# Autodesk Inventor assembly: 01 Gesamtsystem
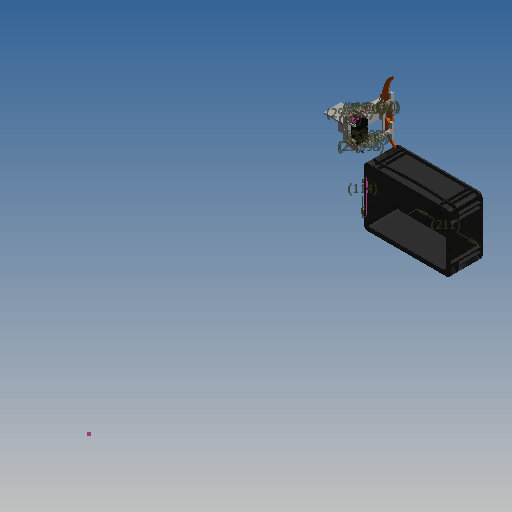
[picture p0: Inventor's stored thumbnail of the model, 512x512]
Saved by Autodesk Inventor 2026.2 (Build 302298000, 298)
## iProperties
Part Number: 01 Gesamtsystem
Document SubType Name: Baugruppe
Designer: Schally
Author: Schally
## Documents named in this file (11)
- E:\06 Carologistics\02 Zeichnungen Greifer System\01 Gesamtsystem.iam
- E:\06 Carologistics\02 Zeichnungen Greifer System\01-01 Gripper_Basis_2 Servo System.ipt
- E:\06 Carologistics\02 Zeichnungen Greifer System\01-02-01 Sandard-Servo.ipt
- E:\06 Carologistics\02 Zeichnungen Greifer System\01-02-03 Gripper neu rechts.ipt
- E:\06 Carologistics\02 Zeichnungen Greifer System\01-03-01 Zange Links.iam
- E:\06 Carologistics\02 Zeichnungen Greifer System\01-03-02 Zange rechts.iam
- E:\06 Carologistics\02 Zeichnungen Greifer System\01-03-05 Muttern.ipt
- E:\06 Carologistics\02 Zeichnungen Greifer System\01-03-06 Schraube unten.ipt
- E:\06 Carologistics\02 Zeichnungen Greifer System\01-05 Absicherung Richtung Kugellager.ipt
- E:\06 Carologistics\02 Zeichnungen Greifer System\00 Zeichnung Box.ipt
- E:\06 Carologistics\02 Zeichnungen Greifer System\01-02-02 Gripper neu links.ipt
## Components (14 placed, 10 different names)
1. 01-01 Gripper_Basis_2 Servo System:1 — Einfügen:1, Passend:1, Passend:20, Passend:21, Passend:22, Passend:23, Passend:24, Passend:25, Passend:28
2. 01-02-01 Sandard-Servo:1 — Passend:20, Passend:21, Passend:22, Passend:26
3. 01-02-03 Gripper neu rechts:1 — Passend:26
4. 01-03-01 Zange Links:1 [sub-assembly] — Passend:3, Passend:5, Passend:9
5. 01-03-02 Zange rechts:1 [sub-assembly] — Passend:2, Passend:10, Passend:11
6. 01-03-05 Muttern:1 — Passend:4, Passend:5
7. 01-03-06 Schraube unten:1 — Einfügen:2, Passend:2, Passend:3, Passend:4, Passend:6, Passend:7, Passend:8, Passend:12
8. 01-05 Absicherung Richtung Kugellager:1 — Einfügen:1, Passend:1, Einfügen:2
9. 01-03-05 Muttern:2 — Passend:8, Passend:11, Passend:12
10. 01-03-05 Muttern:3 — Passend:6, Passend:10, Passend:13
11. 01-03-05 Muttern:4 — Passend:7, Passend:9, Passend:13
12. 00 Zeichnung Box:1 — Passend:28
13. 01-02-01 Sandard-Servo:2 — Passend:23, Passend:24, Passend:25, Passend:27
14. 01-02-02 Gripper neu links:1 — Passend:27
## Relationships (24: Mate 22, Insert 2)
- Einfügen:1 [Insert]: 01-01 Gripper_Basis_2 Servo System:1 ↔ 01-05 Absicherung Richtung Kugellager:1
- Passend:1 [Mate]: 01-01 Gripper_Basis_2 Servo System:1 ↔ 01-05 Absicherung Richtung Kugellager:1
- Einfügen:2 [Insert]: 01-03-06 Schraube unten:1 ↔ 01-05 Absicherung Richtung Kugellager:1
- Passend:2 [Mate]: 01-03-02 Zange rechts:1 ↔ 01-03-06 Schraube unten:1
- Passend:3 [Mate]: 01-03-01 Zange Links:1 ↔ 01-03-06 Schraube unten:1
- Passend:4 [Mate]: 01-03-05 Muttern:1 ↔ 01-03-06 Schraube unten:1
- Passend:5 [Mate]: 01-03-01 Zange Links:1 ↔ 01-03-05 Muttern:1
- Passend:6 [Mate]: 01-03-06 Schraube unten:1 ↔ 01-03-05 Muttern:3
- Passend:7 [Mate]: 01-03-06 Schraube unten:1 ↔ 01-03-05 Muttern:4
- Passend:8 [Mate]: 01-03-06 Schraube unten:1 ↔ 01-03-05 Muttern:2
- Passend:9 [Mate]: 01-03-01 Zange Links:1 ↔ 01-03-05 Muttern:4
- Passend:10 [Mate]: 01-03-02 Zange rechts:1 ↔ 01-03-05 Muttern:3
- Passend:11 [Mate]: 01-03-02 Zange rechts:1 ↔ 01-03-05 Muttern:2
- Passend:12 [Mate]: 01-03-06 Schraube unten:1 ↔ 01-03-05 Muttern:2
- Passend:13 [Mate]: 01-03-05 Muttern:3 ↔ 01-03-05 Muttern:4
- Passend:20 [Mate]: 01-01 Gripper_Basis_2 Servo System:1 ↔ 01-02-01 Sandard-Servo:1
- Passend:21 [Mate]: 01-01 Gripper_Basis_2 Servo System:1 ↔ 01-02-01 Sandard-Servo:1
- Passend:22 [Mate]: 01-01 Gripper_Basis_2 Servo System:1 ↔ 01-02-01 Sandard-Servo:1
- Passend:23 [Mate]: 01-01 Gripper_Basis_2 Servo System:1 ↔ 01-02-01 Sandard-Servo:2
- Passend:24 [Mate]: 01-01 Gripper_Basis_2 Servo System:1 ↔ 01-02-01 Sandard-Servo:2
- Passend:25 [Mate]: 01-01 Gripper_Basis_2 Servo System:1 ↔ 01-02-01 Sandard-Servo:2
- Passend:26 [Mate]: 01-02-01 Sandard-Servo:1 ↔ 01-02-03 Gripper neu rechts:1
- Passend:27 [Mate]: 01-02-01 Sandard-Servo:2 ↔ 01-02-02 Gripper neu links:1
- Passend:28 [Mate]: 01-01 Gripper_Basis_2 Servo System:1 ↔ 00 Zeichnung Box:1
